# Autodesk Inventor assembly: omni-wheel-90deg
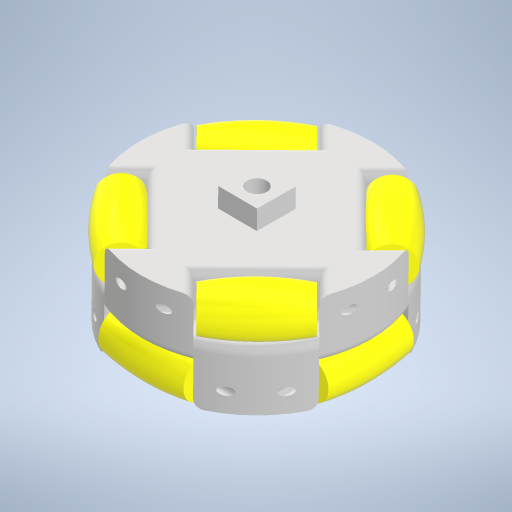
[picture p0: Inventor's stored thumbnail of the model, 512x512]
Saved by Autodesk Inventor 2024.2 (Build 282272000, 272)
## iProperties
Created: 2024-04-01
Part Number: omni-wheel-90deg
Document SubType Name: Assembly
Designer: Robin
Author: Robin
## Documents named in this file (4)
- C:\Users\Robin\Documents\MechanicalDesign\CAD\omni-wheel-90deg.iam
- C:\Users\Robin\Documents\MechanicalDesign\CAD\omni-wheel.ipt
- C:\Users\Robin\Documents\MechanicalDesign\CAD\roller.ipt
- C:\Users\Robin\Documents\MechanicalDesign\CAD\wheel-lock.ipt
## Components (10 placed, 3 different names)
1. omni-wheel:1 — Mate:1, Mate:2, Mate:3, Mate:4, Mate:5, Mate:6, Mate:7, Mate:8, Mate:9, Mate:10, Mate:11, Mate:12, Mate:13, Mate:14, Mate:15, Mate:16, Mate:17, Mate:18, Flush:1
2. roller:1 — Mate:1, Mate:2
3. roller:2 — Mate:3, Mate:4
4. roller:3 — Mate:5, Mate:6
5. roller:4 — Mate:11, Mate:12
6. roller:5 — Mate:9, Mate:10
7. roller:6 — Mate:13, Mate:14
8. roller:7 — Mate:15, Mate:16
9. roller:8 — Mate:7, Mate:8
10. wheel-lock:1 — Mate:17, Mate:18, Flush:1
## Relationships (19: Mate 18, Flush 1)
- Mate:1 (0.5 mm): omni-wheel:1 ↔ roller:1
- Mate:2: omni-wheel:1 ↔ roller:1
- Mate:3: omni-wheel:1 ↔ roller:2
- Mate:4 (0.5 mm): omni-wheel:1 ↔ roller:2
- Mate:5: omni-wheel:1 ↔ roller:3
- Mate:6 (0.5 mm): omni-wheel:1 ↔ roller:3
- Mate:7 (0.5 mm): omni-wheel:1 ↔ roller:8
- Mate:8: omni-wheel:1 ↔ roller:8
- Mate:9 (0.5 mm): omni-wheel:1 ↔ roller:5
- Mate:10: omni-wheel:1 ↔ roller:5
- Mate:11 (0.5 mm): omni-wheel:1 ↔ roller:4
- Mate:12: omni-wheel:1 ↔ roller:4
- Mate:13: omni-wheel:1 ↔ roller:6
- Mate:14 (0.5 mm): omni-wheel:1 ↔ roller:6
- Mate:15: omni-wheel:1 ↔ roller:7
- Mate:16 (0.5 mm): omni-wheel:1 ↔ roller:7
- Mate:17: omni-wheel:1 ↔ wheel-lock:1
- Mate:18: omni-wheel:1 ↔ wheel-lock:1
- Flush:1: omni-wheel:1 ↔ wheel-lock:1
